# Autodesk Inventor assembly: ICF34_70mmNipple
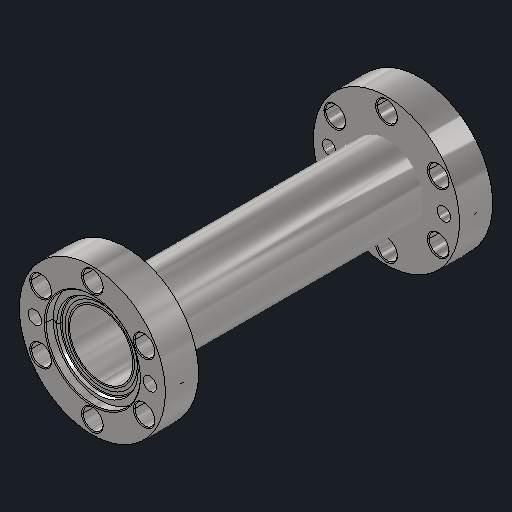
[picture p0: Inventor's stored thumbnail of the model, 512x512]
Saved by Autodesk Inventor 2026 (Build 300175050, 175E)
## iProperties
Created: 2023-07-13
Part Number: ICF34_70mmNipple
Document SubType Name: Assembly
Designer: kuzmin
Author: kuzmin
## Documents named in this file (3)
- C:\Users\queez\Dropbox\Drawings\PIHTI\PALP\CF34-nipples-for-PALP\ICF34_70mmNipple.iam
- C:\Users\queez\Dropbox\Drawings\PIHTI\PALP\CF34-nipples-for-PALP\ICF34_70mmNipplePipe.ipt
- C:\Users\queez\Dropbox\Drawings\PIHTI\PALP\Prototype-PALP-CF34-flange.ipt
## Components (3 placed, 2 different names)
1. ICF34_70mmNipplePipe:1 — Rigid:1, Rotational:3
2. Prototype-PALP-CF34-flange:1 — Rigid:1, Mate:1
3. Prototype-PALP-CF34-flange:2 — Rotational:3, Mate:1
## Relationships (3: WeldJoint 1, RevoluteJoint 1, Mate 1)
- Rigid:1 [WeldJoint]: ICF34_70mmNipplePipe:1 ↔ Prototype-PALP-CF34-flange:1
- Rotational:3 [RevoluteJoint]: ICF34_70mmNipplePipe:1 ↔ Prototype-PALP-CF34-flange:2
- Mate:1: Prototype-PALP-CF34-flange:1 ↔ Prototype-PALP-CF34-flange:2
